# Autodesk Inventor assembly: Battery Bolt
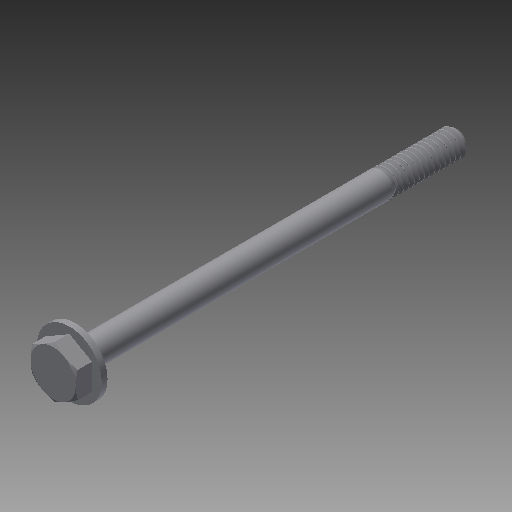
[picture p0: Inventor's stored thumbnail of the model, 512x512]
Saved by Autodesk Inventor 2017 (Build 210142000, 142)
## iProperties
Created: 2022-08-16
Part Number: Battery Bolt
Document SubType Name: Assembly
Designer: JTS
Author: JTS
## Documents named in this file (3)
- C:\Users\Windermac\Desktop\MASTER Honda Insight G1 IMA Bay\Battery Bolt.iam
- C:\Users\Windermac\Desktop\MASTER Honda Insight G1 IMA Bay\Bolt - Hex - 0.250in-20 3.750in 92198A557.ipt
- C:\Users\Windermac\Desktop\MASTER Honda Insight G1 IMA Bay\Washer 0.250in 92141A029.ipt
## Components (2 placed, 2 different names)
1. Bolt - Hex - 0.250in-20 3.750in 92198A557:1 — Insert:1
2. Washer 0.250in 92141A029:1 — Insert:1
## Relationships (1: Insert 1)
- Insert:1: Bolt - Hex - 0.250in-20 3.750in 92198A557:1 ↔ Washer 0.250in 92141A029:1
